# Autodesk Inventor assembly: ABD_MX_64_Slider_Fixation_Set_Left2Horn
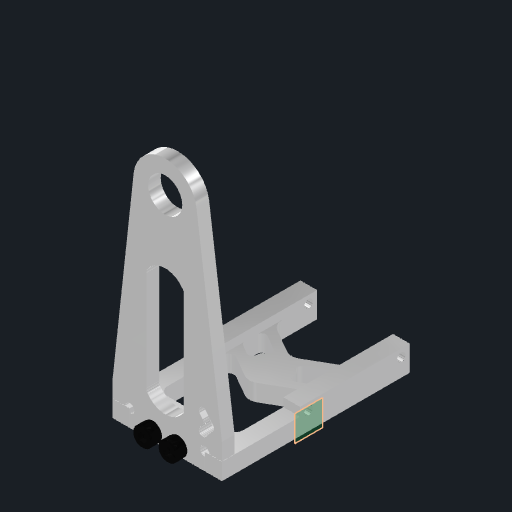
[picture p0: Inventor's stored thumbnail of the model, 512x512]
Saved by Autodesk Inventor 2024.3 (Build 283343000, 343)
## iProperties
Created: 2024-02-15
Part Number: ABD_MX_64_Slider_Fixation_Set_Left2Horn
Document SubType Name: Assembly
Designer: ASUS
Author: ASUS
## Documents named in this file (4)
- C:\Users\ASUS\Desktop\Anti_Backlash_Structure_OP\v2_Frame\ABD_MX_64_Slider_Fixation_Set_Left2Horn.iam
- C:\Users\ASUS\Desktop\Anti_Backlash_Structure_OP\MISUMI\CSH-ST-M2_5-8_203.ipt
- C:\Users\ASUS\Desktop\Anti_Backlash_Structure_OP\v2_Frame\Leg_joint_slider_frame_v2.ipt
- C:\Users\ASUS\Desktop\Anti_Backlash_Structure_OP\v2_Frame\106_Slider_Fixation.ipt
## Components (4 placed, 3 different names)
1. Leg_joint_slider_frame_v2:1 — 메이트:1, 메이트:2, 메이트:3, 삽입:1, 삽입:2
2. 106_Slider_Fixation:1 — 메이트:1, 메이트:2, 메이트:3
3. CSH-ST-M2_5-8_203:1 — 삽입:1
4. CSH-ST-M2_5-8_203:2 — 삽입:2
## Relationships (5: Mate 3, Insert 2)
- 메이트:1 [Mate]: Leg_joint_slider_frame_v2:1 ↔ 106_Slider_Fixation:1
- 메이트:2 [Mate]: Leg_joint_slider_frame_v2:1 ↔ 106_Slider_Fixation:1
- 메이트:3 [Mate]: Leg_joint_slider_frame_v2:1 ↔ 106_Slider_Fixation:1
- 삽입:1 [Insert]: Leg_joint_slider_frame_v2:1 ↔ CSH-ST-M2_5-8_203:1
- 삽입:2 [Insert]: Leg_joint_slider_frame_v2:1 ↔ CSH-ST-M2_5-8_203:2
